# Autodesk Inventor assembly: SOLAR PACKING
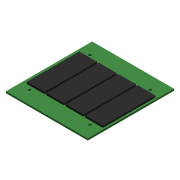
[picture p0: Inventor's stored thumbnail of the model, 180x180]
Saved by Autodesk Inventor 2018 (Build 220112000, 112)
## iProperties
Created: 2018-12-16
Part Number: SOLAR PACKING
Document SubType Name: Assembly
Designer: R.P.SMITH
Mass: 30.7278 g
Surface Area: 311.545 cm^2
Volume: 28.9885 cm^3
Density: 1.06 g/cm^3
Author: R.P.SMITH
## Documents named in this file (3)
- D:\Documents\College\Semesters\4 - Fall\Senior Project 2\CADD Files\SOLAR PACKING.iam
- D:\Documents\College\Semesters\4 - Fall\Senior Project 2\CADD Files\Custom Parts\GENERIC SOLAR PANEL.ipt
- D:\Documents\College\Semesters\4 - Fall\Senior Project 2\CADD Files\Digi-key\SLMD121H09L.ipt
## Components (5 placed, 2 different names)
1. GENERIC SOLAR PANEL:1 — Mate:1, Mate:2, Mate:3, Mate:4, Flush:4, Flush:5
2. SLMD121H09L:1 — Mate:4, Flush:1, Flush:3, Mate:5, Mate:6
3. SLMD121H09L:2 — Mate:3, Flush:3, Mate:5, Flush:4, Flush:5
4. SLMD121H09L:3 — Mate:2, Flush:1, Flush:2, Mate:6, Mate:7
5. SLMD121H09L:4 — Mate:1, Flush:2, Mate:7
## Relationships (12: Mate 7, Flush 5)
- Mate:1: GENERIC SOLAR PANEL:1 ↔ SLMD121H09L:4
- Mate:2: GENERIC SOLAR PANEL:1 ↔ SLMD121H09L:3
- Mate:3: GENERIC SOLAR PANEL:1 ↔ SLMD121H09L:2
- Mate:4: GENERIC SOLAR PANEL:1 ↔ SLMD121H09L:1
- Flush:1: SLMD121H09L:1 ↔ SLMD121H09L:3
- Flush:2: SLMD121H09L:3 ↔ SLMD121H09L:4
- Flush:3: SLMD121H09L:1 ↔ SLMD121H09L:2
- Mate:5 (2 mm): SLMD121H09L:1 ↔ SLMD121H09L:2
- Mate:6 (2 mm): SLMD121H09L:1 ↔ SLMD121H09L:3
- Mate:7 (2 mm): SLMD121H09L:3 ↔ SLMD121H09L:4
- Flush:4 (-2 mm): GENERIC SOLAR PANEL:1 ↔ SLMD121H09L:2
- Flush:5 (19.5 mm): GENERIC SOLAR PANEL:1 ↔ SLMD121H09L:2
## Named parameters: SPACING = 2 mm
